# Autodesk Inventor assembly: Ensamblaje2
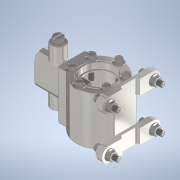
[picture p0: Inventor's stored thumbnail of the model, 180x180]
Saved by Autodesk Inventor 2020 (Build 240168000, 168)
## iProperties
Created: 2020-04-21
Part Number: Ensamblaje2
Document SubType Name: Assembly
Designer: luisg
Author: Luis Gallardo
## Documents named in this file (7)
- C:\Users\luisg\Desktop\Examen Unidad I INVENTOR\Practica 23.7\Ensamblaje2.iam
- C:\Users\luisg\Desktop\Examen Unidad I INVENTOR\Practica 23.7\EXAMEN.ipt
- C:\Users\luisg\Documents\Inventor\Content Center Files\R2020\es-ES\ANSI B 18.6.7 M IFI 513(2)\ANSI B 18.6.7 M _ IFI 513 - M8x1.25 x 30(1).ipt
- C:\Users\luisg\Documents\Inventor\Content Center Files\R2020\es-ES\ANSI B18.6.3(49)\ANSI B18.6.3 - 3_8-16 x 3_8(5).ipt
- C:\Users\luisg\Documents\Inventor\Content Center Files\R2020\es-ES\ISO 4161\ISO 4161 - M8(1).ipt
- C:\Users\luisg\Documents\Inventor\Content Center Files\R2020\es-ES\ANSI B 18.6.7 M IFI 513(3)\ANSI B 18.6.7 M _ IFI 513 - M8x1.25 x 30(2).ipt
- C:\Users\luisg\Documents\Inventor\Content Center Files\R2020\es-ES\AS 1427(02)\AS 1427 - M8 x 80(2).ipt
## Components (18 placed, 6 different names)
1. EXAMEN:1 — Coincidencia:1, Coincidencia:2, Coincidencia:3, Coincidencia:4, Coincidencia:5, Coincidencia:6, Coincidencia:7, Coincidencia:8, Insertar:1, Insertar:2, Insertar:3, Insertar:4, Insertar:5, Insertar:6, Insertar:7, Insertar:8, Insertar:9, Insertar:10, Insertar:11, Insertar:12, Insertar:13
2. Tornillo para maquinaria de cabeza hex. bridada - Métrico M8x1.25 x 30:1 — Coincidencia:1, Coincidencia:2
3. Tornillo para maquinaria de cabeza hex. bridada - Métrico M8x1.25 x 30:2 — Coincidencia:3, Coincidencia:4
4. Tornillo para maquinaria de cabeza hex. bridada - Métrico M8x1.25 x 30:3 — Coincidencia:5, Coincidencia:6
5. Tornillo para maquinaria de cabeza hex. bridada - Métrico M8x1.25 x 30:4 — Coincidencia:7, Coincidencia:8
6. ISO 4161 M8:2 — Insertar:1
7. ISO 4161 M8:3 — Insertar:2
8. ISO 4161 M8:4 — Insertar:3
9. ISO 4161 M8:1 — Insertar:4
10. Tornillo para maquinaria de cabeza hex. bridada dentada - Métrico M8x1.25 x 30:1 — Insertar:5
11. Tornillo para maquinaria de cabeza hex. bridada dentada - Métrico M8x1.25 x 30:2 — Insertar:6
12. Tornillo para maquinaria de cabeza hex. bridada dentada - Métrico M8x1.25 x 30:3 — Insertar:7
13. Tornillo para maquinaria de cabeza hex. bridada dentada - Métrico M8x1.25 x 30:4 — Insertar:8
14. Tornillo para maquinaria de cabeza hex. bridada dentada - Métrico M8x1.25 x 30:5 — Insertar:9
15. Tornillo para maquinaria de cabeza hex. bridada dentada - Métrico M8x1.25 x 30:6 — Insertar:10
16. Tornillo para maquinaria para arandela de cabeza hex. ranurada - Pulgadas 3/8-16x0.375:1 — Insertar:11
17. AS 1427 - Métrico M8 x 80:1 — Insertar:12
18. AS 1427 - Métrico M8 x 80:2 — Insertar:13
## Relationships (21: Insert 13, Mate 8)
- Coincidencia:1 [Mate]: EXAMEN:1 ↔ Tornillo para maquinaria de cabeza hex. bridada - Métrico M8x1.25 x 30:1
- Coincidencia:2 [Mate]: EXAMEN:1 ↔ Tornillo para maquinaria de cabeza hex. bridada - Métrico M8x1.25 x 30:1
- Coincidencia:3 [Mate]: EXAMEN:1 ↔ Tornillo para maquinaria de cabeza hex. bridada - Métrico M8x1.25 x 30:2
- Coincidencia:4 [Mate]: EXAMEN:1 ↔ Tornillo para maquinaria de cabeza hex. bridada - Métrico M8x1.25 x 30:2
- Coincidencia:5 [Mate]: EXAMEN:1 ↔ Tornillo para maquinaria de cabeza hex. bridada - Métrico M8x1.25 x 30:3
- Coincidencia:6 [Mate]: EXAMEN:1 ↔ Tornillo para maquinaria de cabeza hex. bridada - Métrico M8x1.25 x 30:3
- Coincidencia:7 [Mate]: EXAMEN:1 ↔ Tornillo para maquinaria de cabeza hex. bridada - Métrico M8x1.25 x 30:4
- Coincidencia:8 [Mate]: EXAMEN:1 ↔ Tornillo para maquinaria de cabeza hex. bridada - Métrico M8x1.25 x 30:4
- Insertar:1: EXAMEN:1 ↔ ISO 4161 M8:2
- Insertar:2: EXAMEN:1 ↔ ISO 4161 M8:3
- Insertar:3: EXAMEN:1 ↔ ISO 4161 M8:4
- Insertar:4: EXAMEN:1 ↔ ISO 4161 M8:1
- Insertar:5: EXAMEN:1 ↔ Tornillo para maquinaria de cabeza hex. bridada dentada - Métrico M8x1.25 x 30:1
- Insertar:6: EXAMEN:1 ↔ Tornillo para maquinaria de cabeza hex. bridada dentada - Métrico M8x1.25 x 30:2
- Insertar:7: EXAMEN:1 ↔ Tornillo para maquinaria de cabeza hex. bridada dentada - Métrico M8x1.25 x 30:3
- Insertar:8: EXAMEN:1 ↔ Tornillo para maquinaria de cabeza hex. bridada dentada - Métrico M8x1.25 x 30:4
- Insertar:9: EXAMEN:1 ↔ Tornillo para maquinaria de cabeza hex. bridada dentada - Métrico M8x1.25 x 30:5
- Insertar:10: EXAMEN:1 ↔ Tornillo para maquinaria de cabeza hex. bridada dentada - Métrico M8x1.25 x 30:6
- Insertar:11: EXAMEN:1 ↔ Tornillo para maquinaria para arandela de cabeza hex. ranurada - Pulgadas 3/8-16x0.375:1
- Insertar:12: EXAMEN:1 ↔ AS 1427 - Métrico M8 x 80:1
- Insertar:13: EXAMEN:1 ↔ AS 1427 - Métrico M8 x 80:2
